# Autodesk Inventor assembly: shooter
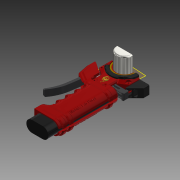
[picture p0: Inventor's stored thumbnail of the model, 180x180]
Saved by Autodesk Inventor 2018 (Build 220112000, 112)
## iProperties
Created: 2019-02-20
Part Number: shooter
Material: 一般
Document SubType Name: Assembly
Designer: ku_sk
Author: ku_sk
## Documents named in this file (15)
- E:\windows\Documents\Inventor\Content Center Files\bay shooter\shooter.iam
- E:\windows\Documents\Inventor\Content Center Files\bay shooter\parts\bay conect.ipt
- E:\windows\Documents\Inventor\Content Center Files\bay shooter\parts\gear.ipt
- E:\windows\Documents\Inventor\Content Center Files\bay shooter\parts\motor.ipt
- E:\windows\Documents\Inventor\Content Center Files\bay shooter\parts\undercover.ipt
- E:\windows\Documents\Inventor\Content Center Files\bay shooter\parts\bearing.ipt
- E:\windows\Documents\Inventor\Content Center Files\bay shooter\parts\battery.ipt
- E:\windows\Documents\Inventor\Content Center Files\bay shooter\parts\brake.ipt
- E:\windows\Documents\Inventor\Content Center Files\bay shooter\parts\bar.ipt
- E:\windows\Documents\Inventor\Content Center Files\bay shooter\parts\switch.ipt
- E:\windows\Documents\Inventor\Content Center Files\bay shooter\parts\joint.ipt
- E:\windows\Documents\Inventor\Content Center Files\bay shooter\parts\circuitcover.ipt
- E:\windows\Documents\Inventor\Content Center Files\bay shooter\parts\circuitcover1.ipt
- E:\windows\Documents\Inventor\Content Center Files\bay shooter\parts\pushbar.ipt
- E:\windows\Documents\Inventor\Content Center Files\bay shooter\parts\toptest.iam
## Components (17 placed, 14 different names)
1. bay conect:1 — メイト:1, フラッシュ:1, メイト:2, メイト:3, メイト:7, メイト:8, メイト:9, メイト:13
2. gear:1 — メイト:2, メイト:3, メイト:5, フラッシュ:5
3. motor:1 — メイト:5, フラッシュ:2, フラッシュ:5, メイト:42
4. undercover:1 — フラッシュ:3, メイト:7, フラッシュ:4, メイト:12, メイト:14, 正接:1, メイト:22, メイト:28, 角度:1, メイト:29, メイト:30, メイト:32, メイト:33, メイト:34, フラッシュ:10, メイト:40, フラッシュ:11
5. bearing:1 — メイト:8, メイト:9, フラッシュ:4
6. battery:1 — メイト:28, 角度:1, メイト:29, メイト:33
7. bar:1 — メイト:13, メイト:14, メイト:15, メイト:24, メイト:41
8. joint:1 — メイト:24, メイト:25
9. circuitcover:1 — メイト:30, メイト:32, メイト:34, メイト:35, フラッシュ:8, フラッシュ:9
10. circuitcover1:1 — メイト:35, フラッシュ:8, フラッシュ:9
11. switch:1 — メイト:22, メイト:25, フラッシュ:10, メイト:37, メイト:38, メイト:39
12. pushbar:1 — メイト:37, メイト:38, メイト:39
13. toptest:1 [sub-assembly] — メイト:40, メイト:41, フラッシュ:11, メイト:42
14. brake:1 — メイト:12, メイト:15, 正接:1
15. brake:2
16. brake:3
17. brake:4
## Component patterns: (4 elements, first: brake:1)
## Relationships (38: Mate 27, Flush 9, Tangent 1, Angle 1)
- メイト:1 [Mate]: bay conect:1
- フラッシュ:1 [Flush]: bay conect:1
- メイト:2 [Mate]: bay conect:1 ↔ gear:1
- メイト:3 [Mate]: bay conect:1 ↔ gear:1
- メイト:5 [Mate]: gear:1 ↔ motor:1
- フラッシュ:2 [Flush]: motor:1
- フラッシュ:3 [Flush]: undercover:1
- メイト:7 [Mate]: bay conect:1 ↔ undercover:1
- メイト:8 [Mate]: bay conect:1 ↔ bearing:1
- メイト:9 [Mate]: bay conect:1 ↔ bearing:1
- フラッシュ:4 [Flush]: undercover:1 ↔ bearing:1
- フラッシュ:5 [Flush]: gear:1 ↔ motor:1
- メイト:12 [Mate] (1.75 mm): undercover:1 ↔ brake:1
- メイト:13 [Mate]: bay conect:1 ↔ bar:1
- メイト:14 [Mate]: undercover:1 ↔ bar:1
- メイト:15 [Mate]: bar:1 ↔ brake:1
- 正接:1 [Tangent]: undercover:1 ↔ brake:1
- メイト:22 [Mate] (0.5 mm): undercover:1 ↔ switch:1
- メイト:24 [Mate]: bar:1 ↔ joint:1
- メイト:25 [Mate]: joint:1 ↔ switch:1
- メイト:28 [Mate]: undercover:1 ↔ battery:1
- 角度:1 [Angle] (0 deg): undercover:1 ↔ battery:1
- メイト:29 [Mate] (-0.5 mm): undercover:1 ↔ battery:1
- メイト:30 [Mate]: undercover:1 ↔ circuitcover:1
- メイト:32 [Mate]: undercover:1 ↔ circuitcover:1
- メイト:33 [Mate] (0.5 mm): undercover:1 ↔ battery:1
- メイト:34 [Mate]: undercover:1 ↔ circuitcover:1
- メイト:35 [Mate]: circuitcover:1 ↔ circuitcover1:1
- フラッシュ:8 [Flush]: circuitcover:1 ↔ circuitcover1:1
- フラッシュ:9 [Flush]: circuitcover:1 ↔ circuitcover1:1
- フラッシュ:10 [Flush] (4.5 mm): undercover:1 ↔ switch:1
- メイト:37 [Mate]: switch:1 ↔ pushbar:1
- メイト:38 [Mate]: switch:1 ↔ pushbar:1
- メイト:39 [Mate]: switch:1 ↔ pushbar:1
- メイト:40 [Mate]: undercover:1 ↔ toptest:1
- メイト:41 [Mate]: bar:1 ↔ toptest:1
- フラッシュ:11 [Flush]: undercover:1 ↔ toptest:1
- メイト:42 [Mate]: motor:1 ↔ toptest:1
